# Autodesk Inventor assembly: Assembly1
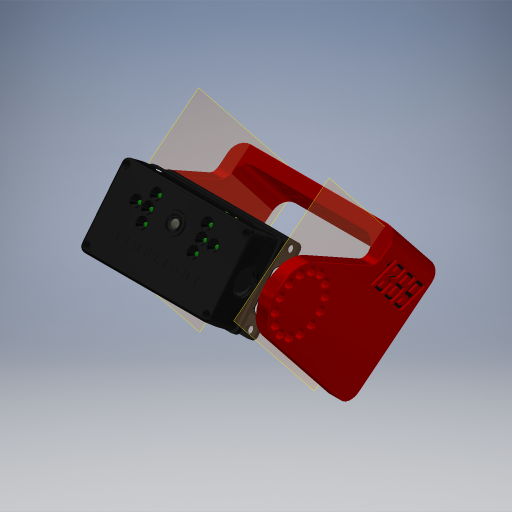
[picture p0: Inventor's stored thumbnail of the model, 512x512]
Saved by Autodesk Inventor 2024.2 (Build 282272000, 272)
## iProperties
Created: 2024-02-01
Part Number: Assembly1
Document SubType Name: Assembly
Designer: rohan
Author: rohan
## Documents named in this file (5)
- C:\Users\rohan\OneDrive - Hillsborough County Public Schools\Robotics\FIRST-Robotics-Competition\Crescendo\Minotaur-Crescendo-Robot\Electronics\Limelight-2-Mount\2024-910-Limelight-2-Mount.iam
- C:\Users\rohan\OneDrive - Hillsborough County Public Schools\Robotics\FIRST-Robotics-Competition\Crescendo\Minotaur-Crescendo-Robot\Electronics\Limelight-2.ipt
- C:\Users\rohan\OneDrive - Hillsborough County Public Schools\Robotics\FIRST-Robotics-Competition\Crescendo\Minotaur-Crescendo-Robot\Electronics\Limelight-2-Mount\2024-900-001-Limelight-Mounting-Plate.ipt
- C:\Users\rohan\OneDrive - Hillsborough County Public Schools\Robotics\FIRST-Robotics-Competition\Crescendo\Minotaur-Crescendo-Robot\Electronics\Limelight-2-Mount\2024-900-002-Thunderhex-Angle-Support.ipt
- C:\Users\rohan\OneDrive - Hillsborough County Public Schools\Robotics\FIRST-Robotics-Competition\Crescendo\Minotaur-Crescendo-Robot\Electronics\Limelight-2-Mount\2024-900-003-Limelight-Extrusion-Mount.ipt
## Components (6 placed, 4 different names)
1. Limelight-2:1 — Mate:1, Insert:1, Insert:2
2. 2024-900-001-Limelight-Mounting-Plate:1 — Mate:1, Insert:1, Insert:2, Mate:2, Mate:3, Mate:5, Mate:6, Symmetry:1, Symmetry:3
3. 2024-900-002-Thunderhex-Angle-Support:3 — Mate:3, Mate:4, Flush:1, Symmetry:2, Symmetry:4, Mate:8
4. 2024-900-002-Thunderhex-Angle-Support:4 — Mate:2, Flush:1, Symmetry:2, Symmetry:4, Mate:7
5. 2024-900-001-Limelight-Mounting-Plate:2 — Mate:4, Mate:5, Mate:6, Symmetry:1, Symmetry:3
6. 2024-900-003-Limelight-Extrusion-Mount:1 — Mate:7, Mate:8
## Relationships (15: Mate 8, Symmetry 4, Insert 2, Flush 1)
- Mate:1: Limelight-2:1 ↔ 2024-900-001-Limelight-Mounting-Plate:1
- Insert:1: Limelight-2:1 ↔ 2024-900-001-Limelight-Mounting-Plate:1
- Insert:2: Limelight-2:1 ↔ 2024-900-001-Limelight-Mounting-Plate:1
- Mate:2: 2024-900-001-Limelight-Mounting-Plate:1 ↔ 2024-900-002-Thunderhex-Angle-Support:4
- Mate:3: 2024-900-001-Limelight-Mounting-Plate:1 ↔ 2024-900-002-Thunderhex-Angle-Support:3
- Mate:4: 2024-900-002-Thunderhex-Angle-Support:3 ↔ 2024-900-001-Limelight-Mounting-Plate:2
- Mate:5: 2024-900-001-Limelight-Mounting-Plate:1 ↔ 2024-900-001-Limelight-Mounting-Plate:2
- Mate:6: 2024-900-001-Limelight-Mounting-Plate:1 ↔ 2024-900-001-Limelight-Mounting-Plate:2
- Flush:1: 2024-900-002-Thunderhex-Angle-Support:3 ↔ 2024-900-002-Thunderhex-Angle-Support:4
- Symmetry:1: 2024-900-001-Limelight-Mounting-Plate:1 ↔ 2024-900-001-Limelight-Mounting-Plate:2
- Symmetry:2: 2024-900-002-Thunderhex-Angle-Support:3 ↔ 2024-900-002-Thunderhex-Angle-Support:4
- Symmetry:3: 2024-900-001-Limelight-Mounting-Plate:1 ↔ 2024-900-001-Limelight-Mounting-Plate:2
- Symmetry:4: 2024-900-002-Thunderhex-Angle-Support:3 ↔ 2024-900-002-Thunderhex-Angle-Support:4
- Mate:7: 2024-900-002-Thunderhex-Angle-Support:4 ↔ 2024-900-003-Limelight-Extrusion-Mount:1
- Mate:8: 2024-900-002-Thunderhex-Angle-Support:3 ↔ 2024-900-003-Limelight-Extrusion-Mount:1
